# Autodesk Inventor assembly: StepperSystem
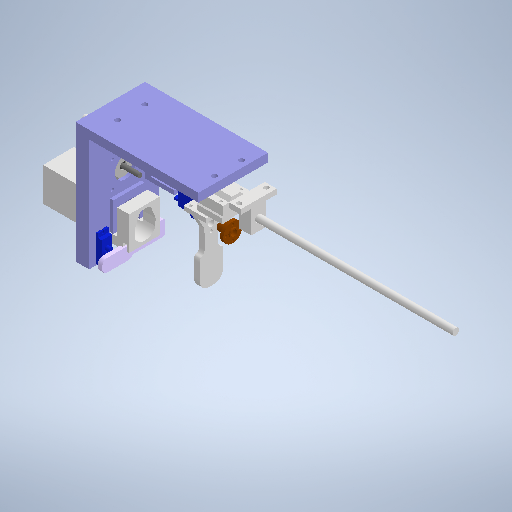
[picture p0: Inventor's stored thumbnail of the model, 512x512]
Saved by Autodesk Inventor 2025.1 (Build 291241000, 241)
## iProperties
Created: 2025-01-26
Part Number: StepperSystem
Document SubType Name: Assembly
Designer: 13156
Author: 13156
## Documents named in this file (12)
- C:\Users\13156\OneDrive - Binghamton University\Documents\GitHub\Perovskite-Automated-Synthesis-System\CAD\Pipette\StepperSystem.iam
- C:\Users\13156\OneDrive - Binghamton University\Documents\GitHub\Perovskite-Automated-Synthesis-System\CAD\Pipette\HolderWStepper.ipt
- C:\Users\13156\OneDrive - Binghamton University\Documents\GitHub\Perovskite-Automated-Synthesis-System\CAD\Non 3D Printed Parts\Linear Rails\8mm Linear Rod.ipt
- C:\Users\13156\OneDrive - Binghamton University\Documents\GitHub\Perovskite-Automated-Synthesis-System\CAD\Non 3D Printed Parts\Linear Rails\Linear Bearing 8mm Square.ipt
- C:\Users\13156\OneDrive - Binghamton University\Documents\GitHub\Perovskite-Automated-Synthesis-System\CAD\Pipette\Actuator.ipt
- C:\Users\13156\OneDrive - Binghamton University\Documents\GitHub\Perovskite-Automated-Synthesis-System\CAD\Pipette\PipetteStand.ipt
- C:\Users\13156\OneDrive - Binghamton University\Documents\GitHub\Perovskite-Automated-Synthesis-System\CAD\Non 3D Printed Parts\Motors and Servos\SG90 Servo.ipt
- C:\Users\13156\OneDrive - Binghamton University\Documents\GitHub\Perovskite-Automated-Synthesis-System\CAD\Pipette\GrabberArm.ipt
- C:\Users\13156\OneDrive - Binghamton University\Documents\GitHub\Perovskite-Automated-Synthesis-System\CAD\Pipette\PipetteSleeve.ipt
- C:\Users\13156\OneDrive - Binghamton University\Documents\GitHub\Perovskite-Automated-Synthesis-System\CAD\Non 3D Printed Parts\Leadscrew.ipt
- C:\Users\13156\OneDrive - Binghamton University\Documents\GitHub\Perovskite-Automated-Synthesis-System\CAD\Non 3D Printed Parts\Linear Rails\Linear Rod Holder SK8.ipt
- C:\Users\13156\OneDrive - Binghamton University\Documents\GitHub\Perovskite-Automated-Synthesis-System\CAD\Non 3D Printed Parts\Motors and Servos\NEMA17 Stepper Motor - 26 mm.ipt
## Components (13 placed, 11 different names)
1. HolderWStepper:1 — Angle:1, Mate:4, Mate:9
2. 8mm Linear Rod:1 — Angle:1, Mate:2
3. Linear Bearing 8mm Square:1 — Mate:2
4. Actuator:1
5. PipetteStand:1 — Mate:7
6. SG90 Servo:1 — Mate:4, Mate:5, Mate:6
7. GrabberArm:1 — Mate:5, Mate:6
8. PipetteSleeve:1 — Mate:7
9. Leadscrew:1
10. Linear Rod Holder SK8:1 — Mate:9
11. Linear Rod Holder SK8:2
12. SG90 Servo:3
13. NEMA17 Stepper Motor - 26 mm:2
## Relationships (7: Mate 6, Angle 1)
- Angle:1 (0 deg): HolderWStepper:1 ↔ 8mm Linear Rod:1
- Mate:2: 8mm Linear Rod:1 ↔ Linear Bearing 8mm Square:1
- Mate:4: HolderWStepper:1 ↔ SG90 Servo:1
- Mate:5: SG90 Servo:1 ↔ GrabberArm:1
- Mate:6: SG90 Servo:1 ↔ GrabberArm:1
- Mate:7: PipetteStand:1 ↔ PipetteSleeve:1
- Mate:9: HolderWStepper:1 ↔ Linear Rod Holder SK8:1
